# Autodesk Inventor assembly: __VK_Indexierung
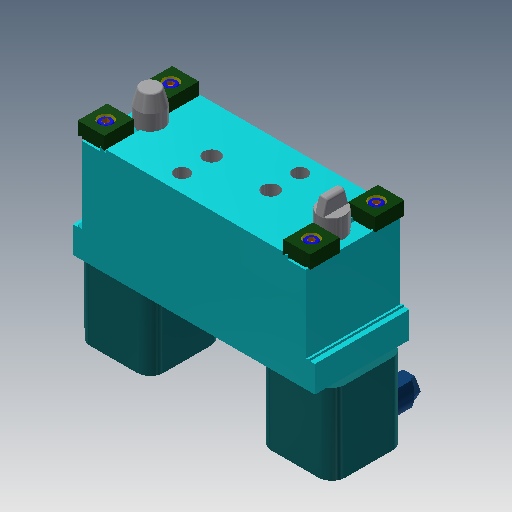
[picture p0: Inventor's stored thumbnail of the model, 512x512]
Saved by Autodesk Inventor 2019 (Build 230136000, 136)
## iProperties
Created: 2023-11-18
Part Number: __VK_Indexierung
Material: Generisch
Document SubType Name: Assembly
Designer: RP
Author: RP
## Documents named in this file (3)
- C:\Users\RP\Documents\Inventor\Projekt_Angelspule\_Verkettung\__VK_Indexierung.iam
- C:\Users\RP\Documents\Inventor\Projekt_Angelspule\_Verkettung\__VK_Indexierung_Basis.ipt
- C:\Users\RP\Documents\Inventor\Projekt_Angelspule\_Verkettung\__VK_Indexierung_Index-Pins.ipt
## Components (2 placed, 2 different names)
1. __VK_Indexierung_Basis:1 — Fluchtend:2, Passend:1, Passend:2, Fluchtend:3, Passend:3, Fluchtend:4
2. __VK_Indexierung_Index-Pins:1 — Passend:1, Passend:2, Fluchtend:3
## Relationships (6: Flush 3, Mate 3)
- Fluchtend:2 [Flush]: __VK_Indexierung_Basis:1
- Passend:1 [Mate]: __VK_Indexierung_Basis:1 ↔ __VK_Indexierung_Index-Pins:1
- Passend:2 [Mate]: __VK_Indexierung_Basis:1 ↔ __VK_Indexierung_Index-Pins:1
- Fluchtend:3 [Flush]: __VK_Indexierung_Basis:1 ↔ __VK_Indexierung_Index-Pins:1
- Passend:3 [Mate]: __VK_Indexierung_Basis:1
- Fluchtend:4 [Flush] (26.0879 mm): __VK_Indexierung_Basis:1
